# Autodesk Inventor assembly: Table Assembly
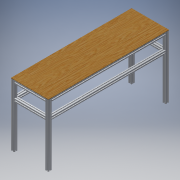
[picture p0: Inventor's stored thumbnail of the model, 180x180]
Saved by Autodesk Inventor 2019.4 (Build 234330000, 330)
## iProperties
Created: 2020-02-27
Part Number: Table Assembly
Document SubType Name: Assembly
Designer: admin
Author: admin
## Documents named in this file (5)
- C:\Users\admin\Desktop\FRC 2020 Engineering\GitHub\7738-2020\Pit Station Designs\Table\Table Assembly.iam
- C:\Users\admin\Desktop\FRC 2020 Engineering\GitHub\7738-2020\Pit Station Designs\Table\Table Leg.ipt
- C:\Users\admin\Desktop\FRC 2020 Engineering\GitHub\7738-2020\Pit Station Designs\Table\Table Leg Struts.ipt
- C:\Users\admin\Desktop\FRC 2020 Engineering\GitHub\7738-2020\Pit Station Designs\Table\Table Leg Struts 2.ipt
- C:\Users\admin\Desktop\FRC 2020 Engineering\GitHub\7738-2020\Pit Station Designs\Table\Table top.ipt
## Components (13 placed, 4 different names)
1. Table Leg:1 — Mate:1, Flush:1, Mate:6, Flush:10, Flush:13, Flush:14, Mate:12, Flush:26
2. Table Leg:2 — Flush:4, Mate:3, Flush:7, Flush:8, Mate:5, Flush:17, Flush:21
3. Table Leg:3 — Flush:3, Mate:4, Flush:5, Flush:6, Mate:8, Flush:15, Flush:16, Flush:19, Mate:9, Mate:10
4. Table Leg:4 — Mate:2, Flush:2, Mate:7, Flush:9, Flush:11, Flush:12, Flush:18, Flush:20, Mate:11
5. Table Leg Struts:1 — Mate:1, Flush:1, Flush:4, Mate:3, Flush:7, Flush:8, Flush:14, Mate:13, Mate:14
6. Table Leg Struts:2 — Mate:2, Flush:2, Flush:3, Mate:4, Flush:5, Flush:6, Flush:11
7. Table Leg Struts 2:1 — Mate:5, Mate:8, Flush:15, Flush:16, Flush:17, Flush:25
8. Table Leg Struts 2:2 — Mate:6, Mate:7, Flush:9, Flush:10, Flush:12, Flush:13
9. Table Leg Struts:3 — Flush:18, Mate:10, Flush:23, Flush:24
10. Table Leg Struts:4 — Flush:21, Mate:12, Mate:13, Flush:22
11. Table Leg Struts 2:3 — Flush:19, Mate:9, Flush:22, Flush:23
12. Table Leg Struts 2:4 — Flush:20, Mate:11, Flush:24
13. Table top:1 — Mate:14, Flush:25, Flush:26
## Relationships (40: Flush 26, Mate 14)
- Mate:1: Table Leg:1 ↔ Table Leg Struts:1
- Flush:1: Table Leg:1 ↔ Table Leg Struts:1
- Mate:2: Table Leg:4 ↔ Table Leg Struts:2
- Flush:2: Table Leg:4 ↔ Table Leg Struts:2
- Flush:3: Table Leg:3 ↔ Table Leg Struts:2
- Flush:4: Table Leg:2 ↔ Table Leg Struts:1
- Mate:3: Table Leg:2 ↔ Table Leg Struts:1
- Mate:4: Table Leg:3 ↔ Table Leg Struts:2
- Flush:5: Table Leg:3 ↔ Table Leg Struts:2
- Flush:6: Table Leg:3 ↔ Table Leg Struts:2
- Flush:7: Table Leg:2 ↔ Table Leg Struts:1
- Flush:8: Table Leg:2 ↔ Table Leg Struts:1
- Mate:5: Table Leg:2 ↔ Table Leg Struts 2:1
- Mate:6: Table Leg:1 ↔ Table Leg Struts 2:2
- Mate:7: Table Leg:4 ↔ Table Leg Struts 2:2
- Flush:9: Table Leg:4 ↔ Table Leg Struts 2:2
- Flush:10: Table Leg:1 ↔ Table Leg Struts 2:2
- Flush:11: Table Leg:4 ↔ Table Leg Struts:2
- Flush:12: Table Leg:4 ↔ Table Leg Struts 2:2
- Flush:13: Table Leg:1 ↔ Table Leg Struts 2:2
- Flush:14: Table Leg:1 ↔ Table Leg Struts:1
- Mate:8: Table Leg:3 ↔ Table Leg Struts 2:1
- Flush:15: Table Leg:3 ↔ Table Leg Struts 2:1
- Flush:16: Table Leg:3 ↔ Table Leg Struts 2:1
- Flush:17: Table Leg:2 ↔ Table Leg Struts 2:1
- Flush:18: Table Leg:4 ↔ Table Leg Struts:3
- Flush:19: Table Leg:3 ↔ Table Leg Struts 2:3
- Flush:20: Table Leg:4 ↔ Table Leg Struts 2:4
- Flush:21: Table Leg:2 ↔ Table Leg Struts:4
- Mate:9: Table Leg:3 ↔ Table Leg Struts 2:3
- Mate:10: Table Leg:3 ↔ Table Leg Struts:3
- Mate:11: Table Leg:4 ↔ Table Leg Struts 2:4
- Mate:12: Table Leg:1 ↔ Table Leg Struts:4
- Mate:13 (150 mm): Table Leg Struts:1 ↔ Table Leg Struts:4
- Flush:22: Table Leg Struts:4 ↔ Table Leg Struts 2:3
- Flush:23: Table Leg Struts:3 ↔ Table Leg Struts 2:3
- Flush:24: Table Leg Struts:3 ↔ Table Leg Struts 2:4
- Mate:14: Table Leg Struts:1 ↔ Table top:1
- Flush:25: Table Leg Struts 2:1 ↔ Table top:1
- Flush:26: Table Leg:1 ↔ Table top:1
